# Autodesk Inventor assembly: final assemblhy explo
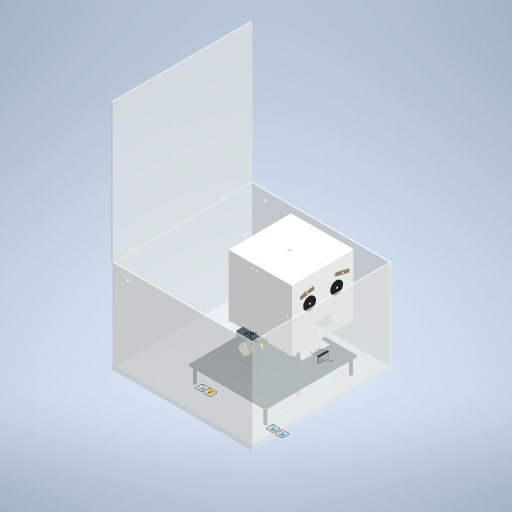
[picture p0: Inventor's stored thumbnail of the model, 512x512]
Saved by Autodesk Inventor 2024 (Build 280153000, 153)
## iProperties
Created: 2023-06-08
Part Number: final assemblhy explo
Document SubType Name: Assembly
Designer: shraa
Author: shraa
## Documents named in this file (5)
- C:\Users\shraa\OneDrive\Documents\explo\final assemblhy explo.iam
- C:\Users\shraa\Downloads\outerboxassembly.iam
- C:\Users\shraa\OneDrive\Documents\explo\bevel mechanism complete.iam
- C:\Users\shraa\Downloads\Face assembly.iam
- C:\Users\shraa\Downloads\toggle switch.iam
## Components (4 placed, 4 different names)
1. outerboxassembly:1 [sub-assembly] — Rotational:1, Rotational:2, Rotational:3, Rigid:1
2. bevel mechanism complete:1 [sub-assembly] — Rotational:1, Rotational:2, Rotational:3, Rotational:4
3. Face assembly:1 [sub-assembly] — Rotational:4
4. toggle switch:1 [sub-assembly] — Rigid:1
## Relationships (5: RevoluteJoint 4, WeldJoint 1)
- Rotational:1 [RevoluteJoint]: outerboxassembly:1 ↔ bevel mechanism complete:1
- Rotational:2 [RevoluteJoint]: outerboxassembly:1 ↔ bevel mechanism complete:1
- Rotational:3 [RevoluteJoint]: outerboxassembly:1 ↔ bevel mechanism complete:1
- Rotational:4 [RevoluteJoint] (100 mm): bevel mechanism complete:1 ↔ Face assembly:1
- Rigid:1 [WeldJoint] (15 mm): outerboxassembly:1 ↔ toggle switch:1
